# Autodesk Inventor assembly: Housing 2
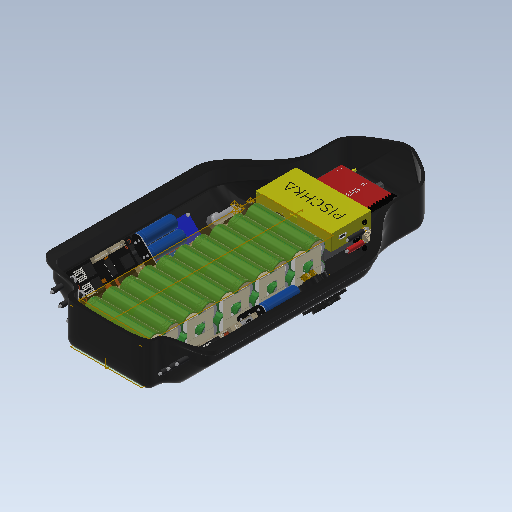
[picture p0: Inventor's stored thumbnail of the model, 512x512]
Saved by Autodesk Inventor 2020.1 (Build 241239000, 239)
## iProperties
Created: 2019-07-14
Part Number: Housing 2
Document SubType Name: Assembly
Designer: Petar
Author: Petar
## Documents named in this file (10)
- D:\OMG\E-Board\CAD\Inventor\Housing\Housing 2.iam
- D:\OMG\E-Board\CAD\Inventor\Electrical Components\Battery Indicator.ipt
- D:\OMG\E-Board\CAD\Inventor\Electrical Components\BMS (separate port).ipt
- D:\OMG\E-Board\CAD\Inventor\Electrical Components\Power Button.ipt
- D:\OMG\E-Board\CAD\Inventor\Electrical Components\VESC - detail.ipt
- D:\OMG\E-Board\CAD\Inventor\Electrical Components\XLR Female Plug.ipt
- D:\OMG\E-Board\CAD\Inventor\Electrical Components\Battery Pack\Samsung 25R\Battery Pack - Samsung 25R - 2xRows.iam
- D:\OMG\E-Board\CAD\Inventor\Housing\Battery Housing.ipt
- D:\OMG\E-Board\CAD\Inventor\Electrical Components\Power Switch - detail.ipt
- D:\OMG\E-Board\CAD\Inventor\Remote\Receiver.iam
## Components (10 placed, 9 different names)
1. Battery Indicator:1 — Rigid:8
2. BMS (separate port):1 — Rigid:3, Rigid:9, Rigid:10
3. Power Button:1 — Rigid:7
4. XLR Female Plug:1 — Rigid:6
5. VESC - detail:1 — Rigid:2
6. VESC - detail:2 — Rigid:1
7. Power Switch - detail:1 — Rigid:10
8. Battery Pack - Samsung 25R - 2xRows:1 [sub-assembly] — Mate:1, Mate:2, Mate:3
9. Battery Housing:1 — Mate:1, Mate:2, Mate:3, Rigid:1, Rigid:2, Rigid:3, Rigid:6, Rigid:8, Rigid:7
10. Receiver:1 [sub-assembly] — Rigid:9
## Relationships (11: WeldJoint 8, Mate 3)
- Mate:1: Battery Pack - Samsung 25R - 2xRows:1 ↔ Battery Housing:1
- Mate:2: Battery Pack - Samsung 25R - 2xRows:1 ↔ Battery Housing:1
- Mate:3: Battery Pack - Samsung 25R - 2xRows:1 ↔ Battery Housing:1
- Rigid:1 [WeldJoint] (6.5 mm): VESC - detail:2 ↔ Battery Housing:1
- Rigid:2 [WeldJoint] (6.5 mm): VESC - detail:1 ↔ Battery Housing:1
- Rigid:3 [WeldJoint]: BMS (separate port):1 ↔ Battery Housing:1
- Rigid:6 [WeldJoint]: XLR Female Plug:1 ↔ Battery Housing:1
- Rigid:7 [WeldJoint] (4 mm): Power Button:1 ↔ Battery Housing:1
- Rigid:8 [WeldJoint]: Battery Indicator:1 ↔ Battery Housing:1
- Rigid:9 [WeldJoint]: BMS (separate port):1 ↔ Receiver:1
- Rigid:10 [WeldJoint] (5 mm): BMS (separate port):1 ↔ Power Switch - detail:1
